# Autodesk Inventor assembly: MechanicalHand
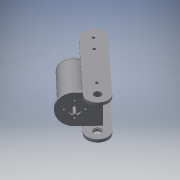
[picture p0: Inventor's stored thumbnail of the model, 180x180]
Saved by Autodesk Inventor 2018 (Build 220112000, 112)
## iProperties
Created: 2017-05-31
Part Number: MechanicalHand
Document SubType Name: Weldment
Designer: Damian
Weld Material: Welded Aluminum-6061
Author: Damian
## Documents named in this file (6)
- C:\Users\Damian\MechanicalHand\CAD\MechanicalHand.iam
- C:\Users\Damian\MechanicalHand\StandardParts\3564_B\3564_B.ipt
- C:\Users\Damian\MechanicalHand\CAD\BaseJointMotorMount.ipt
- C:\Users\Damian\MechanicalHand\CAD\BaseJointPlate.ipt
- C:\Users\Damian\MechanicalHand\CAD\Bushing.ipt
- C:\Users\Damian\MechanicalHand\CAD\BushingLarge.ipt
## Components (6 placed, 5 different names)
1. 3564_B:1 — Mate:1, Mate:2, Mate:3
2. BaseJointMotorMount:1 — Mate:1, Mate:2, Mate:3, Mate:4, Mate:5, Mate:6, Mate:7, Mate:9
3. BaseJointPlate:1 — Mate:4, Mate:5, Mate:11
4. BaseJointPlate:2 — Mate:6, Mate:7, Mate:8, Mate:10, Mate:12
5. Bushing:1 — Mate:8, Mate:9
6. BushingLarge:1 — Mate:10, Mate:11, Mate:12
## Relationships (12: Mate 12)
- Mate:1: 3564_B:1 ↔ BaseJointMotorMount:1
- Mate:2: 3564_B:1 ↔ BaseJointMotorMount:1
- Mate:3: 3564_B:1 ↔ BaseJointMotorMount:1
- Mate:4: BaseJointMotorMount:1 ↔ BaseJointPlate:1
- Mate:5: BaseJointMotorMount:1 ↔ BaseJointPlate:1
- Mate:6: BaseJointMotorMount:1 ↔ BaseJointPlate:2
- Mate:7: BaseJointMotorMount:1 ↔ BaseJointPlate:2
- Mate:8: BaseJointPlate:2 ↔ Bushing:1
- Mate:9: BaseJointMotorMount:1 ↔ Bushing:1
- Mate:10: BaseJointPlate:2 ↔ BushingLarge:1
- Mate:11: BaseJointPlate:1 ↔ BushingLarge:1
- Mate:12: BaseJointPlate:2 ↔ BushingLarge:1
